# Autodesk Inventor assembly: chipshouter_mount_assembly
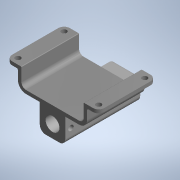
[picture p0: Inventor's stored thumbnail of the model, 180x180]
Saved by Autodesk Inventor 2022 (Build 260153000, 153)
## iProperties
Part Number: chipshouter_mount_assembly
Document SubType Name: Baugruppe
Designer: Niclas
Author: Niclas
## Documents named in this file (4)
- C:\Users\Niclas\Desktop\CAD Files\chipshouter_mount\chipshouter_mount_assembly.iam
- C:\Users\Niclas\Desktop\emfi-main\emfi-main\cad\Workspace\microscope_mount.ipt
- C:\Users\Niclas\Desktop\emfi-main\emfi-main\cad\Workspace\chipshouter_mount_bracket.ipt
- chipshouter_mount_top.ipt
## Components (2 placed, 2 different names)
1. microscope_mount:1 — Passend:1, Fluchtend:1, Fluchtend:2
2. chipshouter_mount_top:1 — Passend:1, Fluchtend:1, Fluchtend:2
## Relationships (3: Flush 2, Mate 1)
- Passend:1 [Mate]: microscope_mount:1 ↔ chipshouter_mount_top:1
- Fluchtend:1 [Flush]: microscope_mount:1 ↔ chipshouter_mount_top:1
- Fluchtend:2 [Flush] (19 mm): microscope_mount:1 ↔ chipshouter_mount_top:1
